# Autodesk Inventor assembly: complete first arm
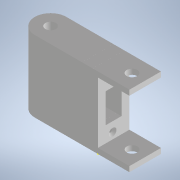
[picture p0: Inventor's stored thumbnail of the model, 180x180]
Saved by Autodesk Inventor 2022 (Build 260153000, 153)
## iProperties
Created: 2021-07-06
Part Number: complete first arm
Document SubType Name: Assembly
Designer: USER
Author: USER
## Documents named in this file (4)
- F:\BVB\robotic arm\complete first arm.iam
- F:\BVB\robotic arm\1st arm.ipt
- F:\BVB\robotic arm\1st arm closing.ipt
- F:\BVB\robotic arm\1st arm to 2nd linking clamp.ipt
## Components (3 placed, 3 different names)
1. 1st arm:1 — Mate:1, Flush:1, Flush:2
2. 1st arm closing:1 — Mate:1, Flush:1, Flush:2, Mate:2, Flush:3, Flush:4
3. 1st arm to 2nd linking clamp:1 — Mate:2, Flush:3, Flush:4
## Relationships (6: Flush 4, Mate 2)
- Mate:1: 1st arm:1 ↔ 1st arm closing:1
- Flush:1: 1st arm:1 ↔ 1st arm closing:1
- Flush:2: 1st arm:1 ↔ 1st arm closing:1
- Mate:2: 1st arm closing:1 ↔ 1st arm to 2nd linking clamp:1
- Flush:3: 1st arm closing:1 ↔ 1st arm to 2nd linking clamp:1
- Flush:4: 1st arm closing:1 ↔ 1st arm to 2nd linking clamp:1
